# Autodesk Inventor assembly: Montagem2
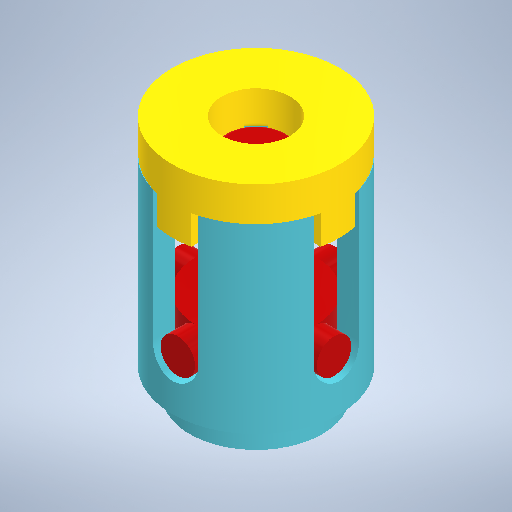
[picture p0: Inventor's stored thumbnail of the model, 512x512]
Saved by Autodesk Inventor 2025.3 (Build 293356000, 356)
## iProperties
Created: 2025-07-28
Part Number: Montagem2
Document SubType Name: Assembly
Designer: user
Author: user
## Documents named in this file (4)
- C:\Users\user\Documents\Inventor\trava_mds\Montagem2.iam
- C:\Users\user\Documents\Inventor\trava_mds\botao.ipt
- C:\Users\user\Documents\Inventor\trava_mds\trava_botao.ipt
- C:\Users\user\Documents\Inventor\trava_mds\trava_botao_topo.ipt
## Components (3 placed, 3 different names)
1. botao:1 — Cilíndrica:1, Rotação/Translação:1, Rotação/Translação:2
2. trava_botao:1 — Cilíndrica:1, Rotação/Translação:1, Rotação/Translação:2, Rígida:1
3. trava_botao_topo:1 — Rígida:1
## Relationships (4: RelateRotateTranslate 2, CylindricalJoint 1, WeldJoint 1)
- Cilíndrica:1 [CylindricalJoint]: botao:1 ↔ trava_botao:1
- Rotação/Translação:1 [RelateRotateTranslate] (12.566 mm): botao:1 ↔ trava_botao:1
- Rotação/Translação:2 [RelateRotateTranslate] (12.566 mm): botao:1 ↔ trava_botao:1
- Rígida:1 [WeldJoint] (-3.8 mm): trava_botao:1 ↔ trava_botao_topo:1
## Named parameters: Finish1_Area = 0.220618, Finish2_Area = 0.220618
note: some values were not read from the file. Shown as the stored number, unit unknown: "Finish1_Area", "Finish2_Area".
